# Autodesk Inventor assembly: Assembly1
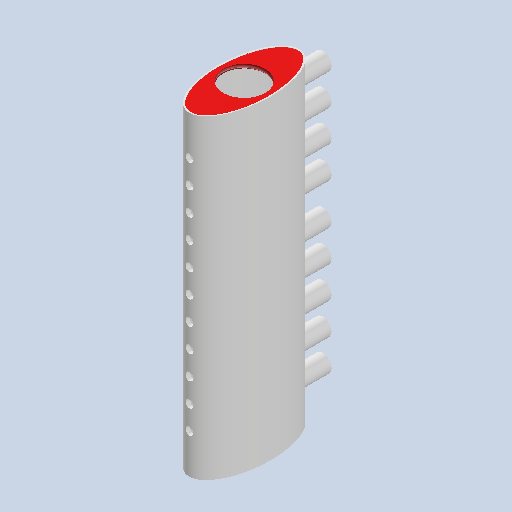
[picture p0: Inventor's stored thumbnail of the model, 512x512]
Saved by Autodesk Inventor 2023 (Build 270158000, 158)
## iProperties
Created: 2022-09-27
Part Number: Assembly1
Document SubType Name: Assembly
Designer: earls
Author: earls
## Documents named in this file (3)
- C:\Users\earls\Documents\stewart-platform\CAD\Smoke generator\Assembly1.iam
- C:\Users\earls\Documents\stewart-platform\CAD\Smoke generator\Smoke visualization device.ipt
- C:\Users\earls\Documents\stewart-platform\CAD\Smoke generator\Smoke visualization bottom.ipt
## Components (2 placed, 2 different names)
1. Smoke visualization device:1 — Mate:1, Mate:2
2. Smoke visualization bottom:1 — Mate:1, Mate:2
## Relationships (2: Mate 2)
- Mate:1: Smoke visualization device:1 ↔ Smoke visualization bottom:1
- Mate:2: Smoke visualization device:1 ↔ Smoke visualization bottom:1
